# Autodesk Inventor assembly: BG001_huenin20_23
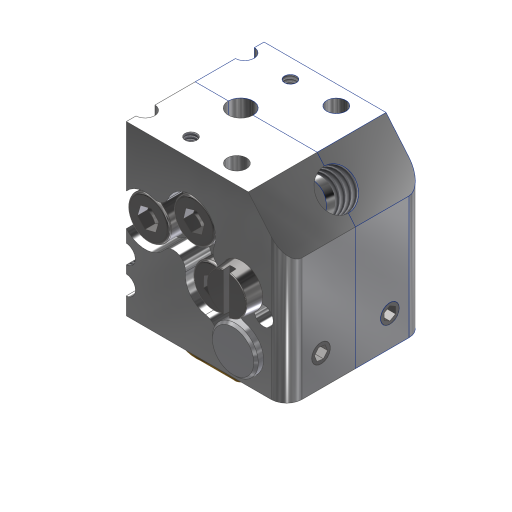
[picture p0: Inventor's stored thumbnail of the model, 512x512]
Saved by Autodesk Inventor 2023.3 (Build 273359000, 359)
## iProperties
Company: HTBLA Kaindorf
RuleStatus: InUse
Created: 2023-08-12
Part Number: BG001_huenin20_23
Project: Fiberprinter-Hotend
Material: Generisch
Description: Fiberprinter_Hotend
Document SubType Name: Assembly
Designer: huenin20
Mass: 129.553 g
Surface Area: 187.581 cm^2
Volume: 21.4141 cm^3
Density: 6.04987 g/cm^3
AfterDocNew0: iProperties-Editor_aufrufen
Author: nicob
Keywords: 2023
## Documents named in this file (21)
- H:\Dokumente\Projects\Kop\Fiberprinter_Hotend\BG001_huenin20_23_Fiberprinter-Hotend_Fiberprinter_Hotend.iam
- H:\Dokumente\Projects\Kop\Fiberprinter_Hotend\Heatingelement.ipt
- H:\Dokumente\Projects\Kop\Fiberprinter_Hotend\BT007_huenin20_23_Fiberprinter-Hotend_Coldend.ipt
- H:\Dokumente\Projects\Kop\Fiberprinter_Hotend\BT001_huenin20_23_Fiberprinter-Hotend_Heizblock_Seite1.ipt
- H:\Dokumente\Projects\Kop\Fiberprinter_Hotend\BT002_huenin20_23_Fiberprinter-Hotend_Heizblock_Seite2.ipt
- H:\Dokumente\Projects\Kop\Fiberprinter_Hotend\BT005_huenin20_23_Fiberprinter-Hotend_Mountingconectors.ipt
- H:\Dokumente\Projects\Kop\Fiberprinter_Hotend\Normteile\de-DE\DIN 912\DIN 912 - M2 x 0,4 x 20 x 19.ipt
- H:\Dokumente\Projects\Kop\Fiberprinter_Hotend\BG004_huenin20_23_Fiberprinter-Hotend_SMN.iam
- H:\Dokumente\Projects\Kop\Fiberprinter_Hotend\Normteile\de-DE\DIN 912\DIN 912 - M3 x 0,5 x 12 x 10,75.ipt
- H:\Dokumente\Projects\Kop\Fiberprinter_Hotend\Step_downloads\Coldend\HeatSink.ipt
- H:\Dokumente\Projects\Kop\Fiberprinter_Hotend\Step_downloads\Bimetal_heatbreak\Bimetal_heatbreak.ipt
- H:\Dokumente\Projects\Kop\Fiberprinter_Hotend\Normteile\de-DE\ISO 1207(1)\DIN EN ISO 1207 - M3 x 4.ipt
- H:\Dokumente\Projects\Kop\Fiberprinter_Hotend\BT009_huenin20_23_Fiberprinter-Hotend_Fiber_führung.ipt
- H:\Dokumente\Projects\Kop\Fiberprinter_Hotend\BG002_huenin20_24_Fiberprinter-Hotend_Nozzel.iam
- H:\Dokumente\Projects\Kop\Fiberprinter_Hotend\Normteile\de-DE\ISO 4026\ISO 4026 - M3 x 3 - ISO.ipt
- H:\Dokumente\Projects\Kop\Fiberprinter_Hotend\BG001_huenin20_23_Fiberprinter-Hotend_Fiberprinter_Hotend\AIP\FEA\ega65v068.fins
- H:\Dokumente\Projects\Kop\Fiberprinter_Hotend\BG001_huenin20_23_Fiberprinter-Hotend_Fiberprinter_Hotend\AIP\FEA\ega65v068.fsat
- H:\Dokumente\Projects\Kop\Fiberprinter_Hotend\BG001_huenin20_23_Fiberprinter-Hotend_Fiberprinter_Hotend\AIP\FEA\ega65v068.ftes
- H:\Dokumente\Projects\Kop\Fiberprinter_Hotend\BG001_huenin20_23_Fiberprinter-Hotend_Fiberprinter_Hotend\AIP\FEA\ega65v068.fwiz
- H:\Dokumente\Projects\Kop\Fiberprinter_Hotend\BG001_huenin20_23_Fiberprinter-Hotend_Fiberprinter_Hotend\AIP\FEA\ega65v0bk.fmsh
- H:\Dokumente\Projects\Kop\Fiberprinter_Hotend\BG001_huenin20_23_Fiberprinter-Hotend_Fiberprinter_Hotend\AIP\FEA\ega65v0bl.fres
## Components (23 placed, 14 different names)
1. BT001_huenin20_23_Fiberprinter-Hotend_Heizblock_Seite1:1 — Einfügen:6, Fluchtend:1, Einfügen:29, Einfügen:30, Einfügen:34, Winkel:1, Einfügen:45, Einfügen:47
2. BT002_huenin20_23_Fiberprinter-Hotend_Heizblock_Seite2:1 — Einfügen:14, Einfügen:15, Fluchtend:2, Passend:1, Einfügen:27, Einfügen:28, Einfügen:38, Einfügen:39, Einfügen:40, Einfügen:44
3. BT007_huenin20_23_Fiberprinter-Hotend_Coldend:1 — Fluchtend:1, Fluchtend:2, Passend:1, Passend:5, Passend:6, Passend:7
4. BG004_huenin20_23_Fiberprinter-Hotend_SMN:1 [sub-assembly] — Passend:5, Passend:6, Einfügen:31, Einfügen:32, Passend:7
5. HeatSink:1 — Einfügen:35, Winkel:1, Einfügen:46
6. Bimetal_heatbreak:1 — Einfügen:34, Einfügen:35
7. BT009_huenin20_23_Fiberprinter-Hotend_Fiber_führung:1 — Einfügen:43
8. BG002_huenin20_24_Fiberprinter-Hotend_Nozzel:1 [sub-assembly] — Einfügen:43, Einfügen:47
9. ISO 4026 M3 x 3:1 — Einfügen:45
10. ISO 4026 M3 x 3:2 — Einfügen:44
11. ISO 4026 M3 x 3:3 — Einfügen:46
12. DIN 912 - ersetzt durch DIN EN ISO 4762 M2 x 20:2 — Einfügen:31
13. BT005_huenin20_23_Fiberprinter-Hotend_Mountingconectors:2 — Einfügen:27
14. BT005_huenin20_23_Fiberprinter-Hotend_Mountingconectors:4 — Einfügen:30
15. BT005_huenin20_23_Fiberprinter-Hotend_Mountingconectors:3 — Einfügen:29
16. BT005_huenin20_23_Fiberprinter-Hotend_Mountingconectors:1 — Einfügen:28
17. DIN 912 - ersetzt durch DIN EN ISO 4762 M2 x 20:1 — Einfügen:32
18. DIN EN ISO 1207 M3 x 4:1 — Einfügen:39
19. DIN 912 - ersetzt durch DIN EN ISO 4762 M3 x 12:2 — Einfügen:14
20. DIN 912 - ersetzt durch DIN EN ISO 4762 M3 x 12:3 — Einfügen:38
21. DIN 912 - ersetzt durch DIN EN ISO 4762 M3 x 12:1 — Einfügen:15
22. DIN EN ISO 1207 M3 x 4:2 — Einfügen:40
23. Heatingelement:1 — Einfügen:6
## Relationships (26: Insert 19, Mate 4, Flush 2, Angle 1)
- Einfügen:6 [Insert] (-1 mm): BT001_huenin20_23_Fiberprinter-Hotend_Heizblock_Seite1:1 ↔ Heatingelement:1
- Einfügen:14 [Insert]: BT002_huenin20_23_Fiberprinter-Hotend_Heizblock_Seite2:1 ↔ DIN 912 - ersetzt durch DIN EN ISO 4762 M3 x 12:2
- Einfügen:15 [Insert]: BT002_huenin20_23_Fiberprinter-Hotend_Heizblock_Seite2:1 ↔ DIN 912 - ersetzt durch DIN EN ISO 4762 M3 x 12:1
- Fluchtend:1 [Flush]: BT001_huenin20_23_Fiberprinter-Hotend_Heizblock_Seite1:1 ↔ BT007_huenin20_23_Fiberprinter-Hotend_Coldend:1
- Fluchtend:2 [Flush] (3 mm): BT002_huenin20_23_Fiberprinter-Hotend_Heizblock_Seite2:1 ↔ BT007_huenin20_23_Fiberprinter-Hotend_Coldend:1
- Passend:1 [Mate] (6 mm): BT002_huenin20_23_Fiberprinter-Hotend_Heizblock_Seite2:1 ↔ BT007_huenin20_23_Fiberprinter-Hotend_Coldend:1
- Einfügen:27 [Insert]: BT002_huenin20_23_Fiberprinter-Hotend_Heizblock_Seite2:1 ↔ BT005_huenin20_23_Fiberprinter-Hotend_Mountingconectors:2
- Einfügen:28 [Insert]: BT002_huenin20_23_Fiberprinter-Hotend_Heizblock_Seite2:1 ↔ BT005_huenin20_23_Fiberprinter-Hotend_Mountingconectors:1
- Einfügen:29 [Insert]: BT001_huenin20_23_Fiberprinter-Hotend_Heizblock_Seite1:1 ↔ BT005_huenin20_23_Fiberprinter-Hotend_Mountingconectors:3
- Einfügen:30 [Insert]: BT001_huenin20_23_Fiberprinter-Hotend_Heizblock_Seite1:1 ↔ BT005_huenin20_23_Fiberprinter-Hotend_Mountingconectors:4
- Passend:5 [Mate]: BT007_huenin20_23_Fiberprinter-Hotend_Coldend:1 ↔ BG004_huenin20_23_Fiberprinter-Hotend_SMN:1
- Passend:6 [Mate]: BT007_huenin20_23_Fiberprinter-Hotend_Coldend:1 ↔ BG004_huenin20_23_Fiberprinter-Hotend_SMN:1
- Einfügen:31 [Insert]: BG004_huenin20_23_Fiberprinter-Hotend_SMN:1 ↔ DIN 912 - ersetzt durch DIN EN ISO 4762 M2 x 20:2
- Einfügen:32 [Insert]: BG004_huenin20_23_Fiberprinter-Hotend_SMN:1 ↔ DIN 912 - ersetzt durch DIN EN ISO 4762 M2 x 20:1
- Passend:7 [Mate]: BT007_huenin20_23_Fiberprinter-Hotend_Coldend:1 ↔ BG004_huenin20_23_Fiberprinter-Hotend_SMN:1
- Einfügen:34 [Insert]: BT001_huenin20_23_Fiberprinter-Hotend_Heizblock_Seite1:1 ↔ Bimetal_heatbreak:1
- Einfügen:35 [Insert]: HeatSink:1 ↔ Bimetal_heatbreak:1
- Winkel:1 [Angle] (90 deg): BT001_huenin20_23_Fiberprinter-Hotend_Heizblock_Seite1:1 ↔ HeatSink:1
- Einfügen:38 [Insert]: BT002_huenin20_23_Fiberprinter-Hotend_Heizblock_Seite2:1 ↔ DIN 912 - ersetzt durch DIN EN ISO 4762 M3 x 12:3
- Einfügen:39 [Insert]: BT002_huenin20_23_Fiberprinter-Hotend_Heizblock_Seite2:1 ↔ DIN EN ISO 1207 M3 x 4:1
- Einfügen:40 [Insert]: BT002_huenin20_23_Fiberprinter-Hotend_Heizblock_Seite2:1 ↔ DIN EN ISO 1207 M3 x 4:2
- Einfügen:43 [Insert] (1 mm): BT009_huenin20_23_Fiberprinter-Hotend_Fiber_führung:1 ↔ BG002_huenin20_24_Fiberprinter-Hotend_Nozzel:1
- Einfügen:44 [Insert]: BT002_huenin20_23_Fiberprinter-Hotend_Heizblock_Seite2:1 ↔ ISO 4026 M3 x 3:2
- Einfügen:45 [Insert]: BT001_huenin20_23_Fiberprinter-Hotend_Heizblock_Seite1:1 ↔ ISO 4026 M3 x 3:1
- Einfügen:46 [Insert]: HeatSink:1 ↔ ISO 4026 M3 x 3:3
- Einfügen:47 [Insert]: BT001_huenin20_23_Fiberprinter-Hotend_Heizblock_Seite1:1 ↔ BG002_huenin20_24_Fiberprinter-Hotend_Nozzel:1
## Named parameters: sa_0 = 3000
note: some values were not read from the file. Shown as the stored number, unit unknown: "sa_0".
